# Autodesk Inventor assembly: custom_chassis
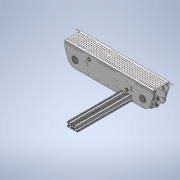
[picture p0: Inventor's stored thumbnail of the model, 180x180]
Saved by Autodesk Inventor 2022 (Build 260153000, 153)
## iProperties
Created: 2021-07-14
Part Number: custom_chassis
Document SubType Name: Assembly
Designer: gfellows
Author: gfellows
## Documents named in this file (17)
- C:\Users\gfellows\Documents\GitHub\8103-CAD-2021-2022\custom_chassis.iam
- C:\Users\gfellows\Documents\GitHub\8103-CAD-2021-2022\outside_plate.ipt
- C:\Users\gfellows\Documents\GitHub\8103-CAD-2021-2022\100 mm mecanum wheel.ipt
- C:\Users\gfellows\Documents\GitHub\8103-CAD-2021-2022\inside_plate.ipt
- C:\Users\gfellows\Documents\GitHub\8103-CAD-2021-2022\1109-0024-0264.ipt
- C:\Users\gfellows\Documents\GitHub\8103-CAD-2021-2022\am-3639 NeveRest Sport, 16-1 with Motor_MIR.ipt
- C:\Users\gfellows\Documents\GitHub\8103-CAD-2021-2022\1611-0514-0006_MIR.ipt
- C:\Users\gfellows\Documents\GitHub\8103-CAD-2021-2022\top_plate.ipt
- C:\Users\gfellows\Documents\GitHub\8103-CAD-2021-2022\6mm axle for bevel gear and pulley.ipt
- C:\Users\gfellows\Documents\GitHub\8103-CAD-2021-2022\0_500_Hex_ID_x_1_125_OD_x_0_313_WD_Flanged_Bearing_v2_217-3875 v1.ipt
- C:\Users\gfellows\Documents\GitHub\8103-CAD-2021-2022\3417-1006-0016 assembly.ipt
- C:\Users\gfellows\Documents\GitHub\8103-CAD-2021-2022\615398 assembly.ipt
- C:\Users\gfellows\Documents\GitHub\8103-CAD-2021-2022\Axle for wheels 1_2_Hex_x_0_201_ID_ThunderHex_Stock_36_217-4017stp.ipt
- C:\Users\gfellows\Documents\GitHub\8103-CAD-2021-2022\spacer_plate.ipt
- C:\Users\gfellows\Documents\GitHub\8103-CAD-2021-2022\wheel_pulley.ipt
- C:\Users\gfellows\Documents\GitHub\8103-CAD-2021-2022\1103-0011-0088.ipt
- C:\Users\gfellows\Documents\GitHub\8103-CAD-2021-2022\2106-4008-0720 assembly.ipt
## Components (41 placed, 16 different names)
1. outside_plate:1 — Cylindrical:1, Cylindrical:2, Flush:3, Flush:6, Angle:2, Rigid:3, Rigid:4, Mate:2, Rigid:6, Rigid:8, Cylindrical:4, Mate:16, Flush:18, Mate:18, Flush:19, Rigid:15, Rigid:16, Rotational:5, Rigid:17
2. 100 mm mecanum wheel:1 — Cylindrical:1, Flush:1
3. 100 mm mecanum wheel:2 — Cylindrical:2, Flush:1, Mate:4
4. inside_plate:1 — Flush:2, Flush:4, Rotational:1, Angle:1, Rotational:2, Rigid:1, Rigid:2, Flush:10, Mate:3, Rigid:7, Rigid:11, Mate:13, Flush:17, Mate:19, Flush:20, Rigid:14, Rigid:18
5. 1109-0024-0264:1 — Rotational:2, Flush:5
6. 1109-0024-0264:2 — Rotational:1, Angle:1, Flush:5
7. am-3639 NeveRest Sport, 16-1 with Motor_MIR:1 — Rigid:10, Rigid:11, Flush:14
8. am-3639 NeveRest Sport, 16-1 with Motor_MIR:2 — Flush:6, Angle:2, Mate:2, Rigid:9
9. 1611-0514-0006_MIR:1 — Rigid:1
10. 1611-0514-0006_MIR:2 — Rigid:2, Cylindrical:5
11. 1611-0514-0006_MIR:3 — Rigid:3, Rotational:3, Cylindrical:3
12. 1611-0514-0006_MIR:4 — Rigid:4, Rotational:4
13. top_plate:1 — Flush:7, Flush:10, Mate:3, Mate:14, Mate:15, Mate:17, Mate:20
14. 6mm axle for bevel gear and pulley:1 — Rotational:3, Cylindrical:6
15. 6mm axle for bevel gear and pulley:2 — Rotational:4
16. 0_500_Hex_ID_x_1_125_OD_x_0_313_WD_Flanged_Bearing_v2_217-3875 v1:1 — Rigid:5, Mate:6
17. 0_500_Hex_ID_x_1_125_OD_x_0_313_WD_Flanged_Bearing_v2_217-3875 v1:2 — Rigid:7, Rigid:13, Flush:12, Mate:8
18. 0_500_Hex_ID_x_1_125_OD_x_0_313_WD_Flanged_Bearing_v2_217-3875 v1:3 — Rigid:8
19. 0_500_Hex_ID_x_1_125_OD_x_0_313_WD_Flanged_Bearing_v2_217-3875 v1:4 — Rigid:6, Rigid:12, Mate:4
20. 3417-1006-0016 assembly:1 — Cylindrical:4, Flush:11
21. 3417-1006-0016 assembly:2 — Cylindrical:3, Flush:11, Flush:12
22. 615398 assembly:1 — Rigid:10
23. 615398 assembly:2 — Cylindrical:6
24. 615398 assembly:3 — Cylindrical:5, Angle:3
25. 615398 assembly:4 — Rigid:9, Angle:3
26. Axle for wheels 1_2_Hex_x_0_201_ID_ThunderHex_Stock_36_217-4017stp:1 — Rigid:12, Mate:5, Mate:7, Rigid:5
27. Axle for wheels 1_2_Hex_x_0_201_ID_ThunderHex_Stock_36_217-4017stp:2 — Rigid:13, Mate:9, Mate:10
28. spacer_plate:1 — Flush:13, Flush:14
29. wheel_pulley:1 — Mate:5, Mate:6, Mate:7
30. wheel_pulley:2 — Mate:8, Mate:9, Mate:10
31. 1103-0011-0088:1 — Mate:13, Mate:14, Flush:17
32. 1103-0011-0088:2 — Mate:15, Mate:16, Flush:18
33. 1103-0011-0088:4 — Mate:17, Mate:18, Flush:19
34. 2106-4008-0720 assembly:1 — Rigid:14
35. 2106-4008-0720 assembly:2 — Rigid:15
36. 2106-4008-0720 assembly:3 — Rigid:16
37. 2106-4008-0720 assembly:4 — Rigid:17
38. 2106-4008-0720 assembly:5 — Rotational:5
39. 2106-4008-0720 assembly:6 — Rigid:18
40. 1103-0011-0088:3 — Mate:19, Flush:20, Mate:20
41. 1103-0011-0088:5
## Component patterns: (2 elements, first: 1103-0011-0088:3)
## Relationships (65: WeldJoint 18, Mate 17, Flush 16, CylindricalJoint 6, RevoluteJoint 5, Angle 3)
- Cylindrical:1: outside_plate:1 ↔ 100 mm mecanum wheel:1
- Cylindrical:2: outside_plate:1 ↔ 100 mm mecanum wheel:2
- Flush:1: 100 mm mecanum wheel:1 ↔ 100 mm mecanum wheel:2
- Flush:2: inside_plate:1
- Flush:3 (72 mm): outside_plate:1
- Flush:4: inside_plate:1
- Rotational:1 [RevoluteJoint]: inside_plate:1 ↔ 1109-0024-0264:2
- Angle:1 (0 deg): inside_plate:1 ↔ 1109-0024-0264:2
- Rotational:2 [RevoluteJoint]: inside_plate:1 ↔ 1109-0024-0264:1
- Flush:5: 1109-0024-0264:1 ↔ 1109-0024-0264:2
- Flush:6: outside_plate:1 ↔ am-3639 NeveRest Sport, 16-1 with Motor_MIR:2
- Angle:2 (0 deg): outside_plate:1 ↔ am-3639 NeveRest Sport, 16-1 with Motor_MIR:2
- Rigid:1 [WeldJoint]: inside_plate:1 ↔ 1611-0514-0006_MIR:1
- Rigid:2 [WeldJoint]: inside_plate:1 ↔ 1611-0514-0006_MIR:2
- Rigid:3 [WeldJoint]: outside_plate:1 ↔ 1611-0514-0006_MIR:3
- Rigid:4 [WeldJoint]: outside_plate:1 ↔ 1611-0514-0006_MIR:4
- Mate:2: outside_plate:1 ↔ am-3639 NeveRest Sport, 16-1 with Motor_MIR:2
- Flush:7: top_plate:1
- Flush:10: inside_plate:1 ↔ top_plate:1
- Mate:3: inside_plate:1 ↔ top_plate:1
- Rotational:3 [RevoluteJoint]: 1611-0514-0006_MIR:3 ↔ 6mm axle for bevel gear and pulley:1
- Rotational:4 [RevoluteJoint]: 1611-0514-0006_MIR:4 ↔ 6mm axle for bevel gear and pulley:2
- Rigid:5 [WeldJoint]: 0_500_Hex_ID_x_1_125_OD_x_0_313_WD_Flanged_Bearing_v2_217-3875 v1:1 ↔ Axle for wheels 1_2_Hex_x_0_201_ID_ThunderHex_Stock_36_217-4017stp:1
- Rigid:6 [WeldJoint]: outside_plate:1 ↔ 0_500_Hex_ID_x_1_125_OD_x_0_313_WD_Flanged_Bearing_v2_217-3875 v1:4
- Rigid:7 [WeldJoint]: inside_plate:1 ↔ 0_500_Hex_ID_x_1_125_OD_x_0_313_WD_Flanged_Bearing_v2_217-3875 v1:2
- Rigid:8 [WeldJoint]: outside_plate:1 ↔ 0_500_Hex_ID_x_1_125_OD_x_0_313_WD_Flanged_Bearing_v2_217-3875 v1:3
- Cylindrical:3: 1611-0514-0006_MIR:3 ↔ 3417-1006-0016 assembly:2
- Cylindrical:4: outside_plate:1 ↔ 3417-1006-0016 assembly:1
- Flush:11: 3417-1006-0016 assembly:1 ↔ 3417-1006-0016 assembly:2
- Rigid:9 [WeldJoint]: am-3639 NeveRest Sport, 16-1 with Motor_MIR:2 ↔ 615398 assembly:4
- Cylindrical:5: 1611-0514-0006_MIR:2 ↔ 615398 assembly:3
- Angle:3 (90 deg): 615398 assembly:3 ↔ 615398 assembly:4
- Rigid:10 [WeldJoint]: am-3639 NeveRest Sport, 16-1 with Motor_MIR:1 ↔ 615398 assembly:1
- Cylindrical:6: 6mm axle for bevel gear and pulley:1 ↔ 615398 assembly:2
- Rigid:11 [WeldJoint] (6.35 mm): inside_plate:1 ↔ am-3639 NeveRest Sport, 16-1 with Motor_MIR:1
- Rigid:12 [WeldJoint] (1 mm): 0_500_Hex_ID_x_1_125_OD_x_0_313_WD_Flanged_Bearing_v2_217-3875 v1:4 ↔ Axle for wheels 1_2_Hex_x_0_201_ID_ThunderHex_Stock_36_217-4017stp:1
- Mate:4 (1 mm): 100 mm mecanum wheel:2 ↔ 0_500_Hex_ID_x_1_125_OD_x_0_313_WD_Flanged_Bearing_v2_217-3875 v1:4
- Rigid:13 [WeldJoint] (2 mm): 0_500_Hex_ID_x_1_125_OD_x_0_313_WD_Flanged_Bearing_v2_217-3875 v1:2 ↔ Axle for wheels 1_2_Hex_x_0_201_ID_ThunderHex_Stock_36_217-4017stp:2
- Flush:12: 0_500_Hex_ID_x_1_125_OD_x_0_313_WD_Flanged_Bearing_v2_217-3875 v1:2 ↔ 3417-1006-0016 assembly:2
- Flush:13: spacer_plate:1
- Flush:14: am-3639 NeveRest Sport, 16-1 with Motor_MIR:1 ↔ spacer_plate:1
- Mate:5: Axle for wheels 1_2_Hex_x_0_201_ID_ThunderHex_Stock_36_217-4017stp:1 ↔ wheel_pulley:1
- Mate:6: 0_500_Hex_ID_x_1_125_OD_x_0_313_WD_Flanged_Bearing_v2_217-3875 v1:1 ↔ wheel_pulley:1
- Mate:7: Axle for wheels 1_2_Hex_x_0_201_ID_ThunderHex_Stock_36_217-4017stp:1 ↔ wheel_pulley:1
- Mate:8: 0_500_Hex_ID_x_1_125_OD_x_0_313_WD_Flanged_Bearing_v2_217-3875 v1:2 ↔ wheel_pulley:2
- Mate:9: Axle for wheels 1_2_Hex_x_0_201_ID_ThunderHex_Stock_36_217-4017stp:2 ↔ wheel_pulley:2
- Mate:10: Axle for wheels 1_2_Hex_x_0_201_ID_ThunderHex_Stock_36_217-4017stp:2 ↔ wheel_pulley:2
- Mate:13: inside_plate:1 ↔ 1103-0011-0088:1
- Mate:14: top_plate:1 ↔ 1103-0011-0088:1
- Flush:17: inside_plate:1 ↔ 1103-0011-0088:1
- Mate:15: top_plate:1 ↔ 1103-0011-0088:2
- Mate:16: outside_plate:1 ↔ 1103-0011-0088:2
- Flush:18: outside_plate:1 ↔ 1103-0011-0088:2
- Mate:17: top_plate:1 ↔ 1103-0011-0088:4
- Mate:18: outside_plate:1 ↔ 1103-0011-0088:4
- Flush:19: outside_plate:1 ↔ 1103-0011-0088:4
- Mate:19: inside_plate:1 ↔ 1103-0011-0088:3
- Flush:20: inside_plate:1 ↔ 1103-0011-0088:3
- Mate:20: top_plate:1 ↔ 1103-0011-0088:3
- Rigid:14 [WeldJoint]: inside_plate:1 ↔ 2106-4008-0720 assembly:1
- Rigid:15 [WeldJoint]: outside_plate:1 ↔ 2106-4008-0720 assembly:2
- Rigid:16 [WeldJoint]: outside_plate:1 ↔ 2106-4008-0720 assembly:3
- Rotational:5 [RevoluteJoint]: outside_plate:1 ↔ 2106-4008-0720 assembly:5
- Rigid:17 [WeldJoint]: outside_plate:1 ↔ 2106-4008-0720 assembly:4
- Rigid:18 [WeldJoint]: inside_plate:1 ↔ 2106-4008-0720 assembly:6
